# Autodesk Inventor assembly: one side of drive
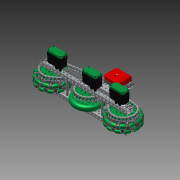
[picture p0: Inventor's stored thumbnail of the model, 180x180]
Saved by Autodesk Inventor 2014 SP1 (Build 180222100, 222)
## iProperties
Created: 2014-03-07
Part Number: one side of drive
Document SubType Name: Assembly
Designer: Ryan
Author: Ryan
## Documents named in this file (25)
- C:\Users\Ryan\Desktop\sw\toss up 5th A bot\drive\one side of drive.iam
- C:\Users\Ryan\Desktop\sw\lib\Aperture VEX CAD Library\Metal\C Channel\2 x 25.ipt
- C:\Users\Ryan\Desktop\sw\lib\Aperture VEX CAD Library\Bearing Blocks\Bearing Block with screws.iam
- C:\Users\Ryan\Desktop\sw\toss up 5th A bot\drive\wheel assembly.iam
- C:\Users\Ryan\Desktop\sw\toss up 5th A bot\drive\varsity wheel with sprocket.iam
- C:\Users\Ryan\Desktop\sw\lib\Aperture VEX CAD Library\Standoffs\BEAM-2000.ipt
- C:\Users\Ryan\Desktop\sw\lib\Aperture VEX CAD Library\Metal\C Channel\5 x 5.ipt
- C:\Users\Ryan\Desktop\sw\lib\Super Sonic Sparks VEX CAD Library\Motors & Sensors\Optical Shaft (Quadrature) Encoder.iam
- C:\Users\Ryan\Desktop\sw\lib\Aperture VEX CAD Library\Spacers\SPACER-0500-0125.ipt
- C:\Users\Ryan\Desktop\sw\lib\Aperture VEX CAD Library\Hardware\8-32\8-32_.375.ipt
- C:\Users\Ryan\Desktop\sw\lib\Aperture VEX CAD Library\Hardware\8-32\8-32 nylock.ipt
- C:\Users\Ryan\Desktop\sw\lib\Aperture VEX CAD Library\Hardware\8-32\8-32_1.500.ipt
- C:\Users\Ryan\Desktop\sw\lib\Aperture VEX CAD Library\Spacers\SPACER-0500-0500.ipt
- C:\Users\Ryan\Desktop\sw\lib\Aperture VEX CAD Library\Spacers\SPACER-0500-0375.ipt
- C:\Users\Ryan\Desktop\sw\lib\Aperture VEX CAD Library\Sprockets\green\High Strength 12-Tooth Sprocket.ipt
- C:\Users\Ryan\Desktop\sw\lib\Aperture VEX CAD Library\Bearing Blocks\Bearing Block.ipt
- C:\Users\Ryan\Desktop\sw\lib\Aperture VEX CAD Library\Hardware\8-32\8-32_.500.ipt
- C:\Users\Ryan\Desktop\sw\lib\Aperture VEX CAD Library\Hardware\Shaft Collar.ipt
- C:\Users\Ryan\Desktop\sw\lib\Aperture VEX CAD Library\Bearing Blocks\Pillow Block.ipt
- C:\Users\Ryan\Desktop\sw\lib\Aperture VEX CAD Library\Spacers\thin\SPACER-0320-0125.ipt
- C:\Users\Ryan\Desktop\sw\lib\Super Sonic Sparks VEX CAD Library\Motors & Sensors\2-Wire Motor 393-Without Wire.iam
- C:\Users\Ryan\Desktop\sw\lib\Aperture VEX CAD Library\Hardware\6-32\6-32_.250.ipt
- C:\Users\Ryan\Desktop\sw\lib\Aperture VEX CAD Library\Shaft\3.7 in shaft.ipt
- C:\Users\Ryan\Desktop\sw\lib\Aperture VEX CAD Library\Sprockets\HS Sprockets\High strength Chain Link.ipt
- C:\Users\Ryan\Desktop\sw\toss up 5th A bot\drive\one side of drive\Design Accelerator\V-Belt transmission1.iam
## Components (178 placed, 24 different names)
1. 2 x 25:1 — Mate:1, Mate:2, Mate:3, Mate:4, Mate:11, Mate:12, Mate:13, Mate:14, Mate:15, Mate:16, Flush:1, Flush:2, Mate:104, Angle:1, Mate:105, Mate:118, Mate:120, Mate:124, Mate:125
2. wheel assembly:1 [sub-assembly] — Mate:5, Mate:20, Mate:92
3. wheel assembly:2 [sub-assembly] — Mate:7, Mate:18, Mate:78
4. varsity wheel with sprocket:1 [sub-assembly] — Mate:10, Mate:19, Flush:4
5. BEAM-2000:1 — Mate:11, Mate:12, Mate:13, Mate:115, Mate:117
6. BEAM-2000:2 — Mate:14, Mate:15, Mate:16, Mate:17, Mate:119, Mate:121
7. 2 x 25:2 — Mate:17, Flush:1, Flush:2, Flush:3, Mate:77, Mate:79, Mate:80, Mate:84, Mate:86, Mate:88, Mate:89, Mate:90, Mate:91, Mate:93, Mate:95, Mate:97, Mate:101, Mate:102, Flush:5, Mate:106, Mate:107, Mate:108, Mate:109, Mate:110, Mate:111, Mate:113, Mate:116, Mate:122, Mate:127, Mate:128, Mate:129, Mate:133
8. 5 x 5:1 — Flush:3, Mate:22, Mate:23, Mate:24, Mate:26, Mate:27, Mate:31, Mate:34, Mate:36, Mate:41, Mate:45, Mate:47, Mate:49, Mate:102, Flush:5, Angle:2
9. Optical Shaft (Quadrature) Encoder:1 [sub-assembly] — Mate:22, Mate:23, Mate:24, Mate:25, Mate:33, Mate:44, Mate:46, Mate:136, Flush:7, Mate:137
10. 8-32_1.500:1 — Mate:34, Mate:36, Mate:42, Mate:43
11. SPACER-0500-0500:1 — Mate:37, Mate:38, Mate:39, Mate:43
12. SPACER-0500-0500:2 — Mate:37, Mate:38, Mate:40
13. SPACER-0500-0375:1 — Mate:39, Mate:40, Mate:41, Mate:42
14. High Strength 12-Tooth Sprocket:1 — Mate:44, Flush:4, Mate:52, Mate:53, Mate:139
15. Bearing Block:1 — Mate:45, Mate:46, Mate:47, Mate:48, Mate:50, Mate:75
16. Shaft Collar:1 — Mate:52, Mate:53, Mate:54, Mate:55
17. SPACER-0500-0500:3 — Mate:54, Mate:55, Mate:56, Mate:57, Mate:76
18. SPACER-0500-0500:4 — Mate:56, Mate:57, Mate:58, Mate:61, Mate:62
19. Pillow Block:1 — Mate:58, Mate:70, Mate:71, Mate:72, Mate:103, Angle:1, Mate:105
20. SPACER-0320-0125:1 — Mate:61, Mate:62, Mate:63, Mate:64
21. SPACER-0320-0125:2 — Mate:63, Mate:64
22. SPACER-0500-0375:2 — Mate:75, Mate:76
23. 2-Wire Motor 393-Without Wire:1 [sub-assembly] — Mate:84, Mate:85, Mate:86, Mate:87
24. Bearing Block:2 — Mate:77, Mate:78, Mate:79, Mate:81, Mate:83, Mate:85
25. 8-32_.375:6 — Mate:106, Mate:107, Mate:108, Mate:114
26. 8-32_.375:7 — Mate:109, Mate:110, Mate:111, Mate:112
27. 8-32 nylock:16 — Mate:112, Mate:113, Flush:6
28. 8-32 nylock:17 — Mate:114, Flush:6
29. 8-32_.375:8 — Mate:115, Mate:116
30. 8-32_.375:9 — Mate:117, Mate:118
31. 8-32_.375:10 — Mate:119, Mate:120
32. 8-32_.375:11 — Mate:121, Mate:122
33. 3.7 in shaft:1 — Mate:136, Flush:7, Mate:137
34. V-Belt transmission:1 [sub-assembly]
35. Bearing Block with screws:1 [sub-assembly] — Mate:1, Mate:2, Mate:3, Mate:4, Mate:5, Mate:20, Mate:123, Mate:126
36. 8-32 nylock:19 — Mate:125, Mate:126
37. 8-32 nylock:18 — Mate:123, Mate:124
38. Bearing Block with screws:2 [sub-assembly] — Mate:10, Mate:19
39. 8-32 nylock:20
40. 8-32 nylock:22
41. Bearing Block with screws:3 [sub-assembly] — Mate:7, Mate:18
42. 8-32 nylock:21
43. 8-32 nylock:23
44. SPACER-0500-0125:1 — Mate:25, Mate:26, Mate:27, Mate:30, Mate:32
45. 8-32_.375:2 — Mate:30, Mate:31
46. 8-32 nylock:1 — Mate:32, Mate:33
47. SPACER-0500-0125:2
48. 8-32_.375:3
49. 8-32 nylock:2
50. 8-32_.500:1 — Mate:48, Mate:49, Mate:51
51. 8-32 nylock:3 — Mate:50, Mate:51
52. 8-32_.500:2
53. 8-32 nylock:4
54. 8-32_.500:3 — Mate:80, Mate:81, Mate:82
55. 8-32 nylock:7 — Mate:82, Mate:83
56. 6-32_.250:1 — Mate:87, Mate:88
57. 8-32_.500:4
58. 8-32 nylock:8
59. 6-32_.250:2
60. 8-32_.375:4 — Mate:71, Mate:72
61. SPACER-0500-0500:6 — Mate:65, Mate:66, Mate:103
62. SPACER-0500-0500:7 — Mate:65, Mate:66, Mate:67, Mate:68, Mate:70
63. SPACER-0500-0500:5 — Mate:67, Mate:68, Mate:74
64. 8-32 nylock:5 — Mate:74, Mate:104
65. 8-32_.375:5
66. SPACER-0500-0500:8
67. SPACER-0500-0500:9
68. SPACER-0500-0500:10
69. 8-32 nylock:13
70. 2-Wire Motor 393-Without Wire:3 [sub-assembly] — Mate:93, Mate:94, Mate:95, Mate:100
71. Bearing Block:4 — Mate:89, Mate:90, Mate:91, Mate:92, Mate:94, Mate:96, Mate:98
72. 2-Wire Motor 393-Without Wire:4 [sub-assembly]
73. Bearing Block:5
74. 8-32_.375:12 — Mate:127, Mate:128, Mate:129
75. 8-32_.375:13 — Mate:134, Mate:135
76. SPACER-0500-0375:4 — Mate:134, Mate:135
77. SPACER-0500-0375:3 — Mate:133
78. 8-32_.375:14
79. 8-32_.375:15
80. SPACER-0500-0375:5
81. SPACER-0500-0375:6
82. High strength Chain Link:1 — Mate:139, Angle:2
83. High strength Chain Link:2
84. High strength Chain Link:3
85. High strength Chain Link:4
86. High strength Chain Link:5
87. High strength Chain Link:6
88. High strength Chain Link:7
89. High strength Chain Link:8
90. High strength Chain Link:9
91. High strength Chain Link:10
92. High strength Chain Link:11
93. High strength Chain Link:12
94. High strength Chain Link:13
95. High strength Chain Link:14
96. High strength Chain Link:15
97. High strength Chain Link:16
98. High strength Chain Link:17
99. High strength Chain Link:18
100. High strength Chain Link:19
101. High strength Chain Link:20
102. High strength Chain Link:21
103. High strength Chain Link:22
104. High strength Chain Link:23
105. High strength Chain Link:24
106. High strength Chain Link:25
107. High strength Chain Link:26
108. High strength Chain Link:27
109. High strength Chain Link:28
110. High strength Chain Link:29
111. High strength Chain Link:30
112. High strength Chain Link:31
113. High strength Chain Link:32
114. High strength Chain Link:33
115. High strength Chain Link:34
116. High strength Chain Link:35
117. High strength Chain Link:36
118. High strength Chain Link:37
119. High strength Chain Link:38
120. High strength Chain Link:39
121. High strength Chain Link:40
122. High strength Chain Link:41
123. High strength Chain Link:42
124. High strength Chain Link:43
125. High strength Chain Link:44
126. High strength Chain Link:45
127. High strength Chain Link:46
128. High strength Chain Link:47
129. High strength Chain Link:48
130. High strength Chain Link:49
131. High strength Chain Link:50
132. High strength Chain Link:51
133. High strength Chain Link:52
134. High strength Chain Link:53
135. High strength Chain Link:54
136. High strength Chain Link:55
137. High strength Chain Link:56
138. High strength Chain Link:57
139. High strength Chain Link:58
140. High strength Chain Link:59
141. High strength Chain Link:60
142. High strength Chain Link:61
143. High strength Chain Link:62
144. High strength Chain Link:63
145. High strength Chain Link:64
146. High strength Chain Link:65
147. High strength Chain Link:66
148. High strength Chain Link:67
149. High strength Chain Link:68
150. High strength Chain Link:69
151. High strength Chain Link:70
152. High strength Chain Link:71
153. High strength Chain Link:72
154. High strength Chain Link:73
155. High strength Chain Link:74
156. High strength Chain Link:75
157. High strength Chain Link:76
158. High strength Chain Link:77
159. High strength Chain Link:78
160. High strength Chain Link:79
161. High strength Chain Link:80
162. High strength Chain Link:81
163. High strength Chain Link:82
164. High strength Chain Link:83
165. High strength Chain Link:84
166. High strength Chain Link:85
167. 6-32_.250:5 — Mate:100, Mate:101
168. 8-32 nylock:11 — Mate:98, Mate:99
169. 8-32_.500:7 — Mate:96, Mate:97, Mate:99
170. 6-32_.250:6
171. 8-32 nylock:12
172. 8-32_.500:8
173. 6-32_.250:7
174. 8-32 nylock:14
175. 8-32_.500:9
176. 6-32_.250:8
177. 8-32 nylock:15
178. 8-32_.500:10
## Component patterns: (3 elements, first: Bearing Block with screws:1 + 8-32 nylock:19 + 8-32 nylock:18), (2 elements, first: SPACER-0500-0125:1 + 8-32_.375:2 + 8-32 nylock:1), (2 elements, first: 8-32_.500:1 + 8-32 nylock:3), (2 elements, first: 8-32_.500:3 + 8-32 nylock:7 + 6-32_.250:1), (2 elements, first: 8-32_.375:4 + SPACER-0500-0500:6 + SPACER-0500-0500:7 + SPACER-0500-0500:5 + 8-32 nylock:5), (2 elements, first: 2-Wire Motor 393-Without Wire:3 + Bearing Block:4), (2 elements, first: 8-32_.375:12 + 8-32_.375:13 + SPACER-0500-0375:4 + SPACER-0500-0375:3), (85 elements, first: High strength Chain Link:1), (2 elements, first: 6-32_.250:5 + 8-32 nylock:11 + 8-32_.500:7), Component Pattern 7:2 (2 elements)
## Relationships (136: Mate 127, Flush 7, Angle 2)
- Mate:1: 2 x 25:1 ↔ Bearing Block with screws:1
- Mate:2 (2.3114 mm): 2 x 25:1 ↔ Bearing Block with screws:1
- Mate:3 (2.3114 mm): 2 x 25:1 ↔ Bearing Block with screws:1
- Mate:4 (2.3114 mm): 2 x 25:1 ↔ Bearing Block with screws:1
- Mate:5: wheel assembly:1 ↔ Bearing Block with screws:1
- Mate:7: wheel assembly:2 ↔ Bearing Block with screws:3
- Mate:10: varsity wheel with sprocket:1 ↔ Bearing Block with screws:2
- Mate:11: 2 x 25:1 ↔ BEAM-2000:1
- Mate:12 (2.3114 mm): 2 x 25:1 ↔ BEAM-2000:1
- Mate:13 (2.3114 mm): 2 x 25:1 ↔ BEAM-2000:1
- Mate:14: 2 x 25:1 ↔ BEAM-2000:2
- Mate:15 (2.3114 mm): 2 x 25:1 ↔ BEAM-2000:2
- Mate:16 (2.3114 mm): 2 x 25:1 ↔ BEAM-2000:2
- Mate:17: BEAM-2000:2 ↔ 2 x 25:2
- Flush:1: 2 x 25:1 ↔ 2 x 25:2
- Mate:18: wheel assembly:2 ↔ Bearing Block with screws:3
- Mate:19: varsity wheel with sprocket:1 ↔ Bearing Block with screws:2
- Mate:20: wheel assembly:1 ↔ Bearing Block with screws:1
- Flush:2: 2 x 25:1 ↔ 2 x 25:2
- Flush:3: 2 x 25:2 ↔ 5 x 5:1
- Mate:22 (2.3114 mm): 5 x 5:1 ↔ Optical Shaft (Quadrature) Encoder:1
- Mate:23 (3.175 mm): 5 x 5:1 ↔ Optical Shaft (Quadrature) Encoder:1
- Mate:24 (-10.3886 mm): 5 x 5:1 ↔ Optical Shaft (Quadrature) Encoder:1
- Mate:25: Optical Shaft (Quadrature) Encoder:1 ↔ SPACER-0500-0125:1
- Mate:26 (2.3114 mm): 5 x 5:1 ↔ SPACER-0500-0125:1
- Mate:27 (2.3114 mm): 5 x 5:1 ↔ SPACER-0500-0125:1
- Mate:30: SPACER-0500-0125:1 ↔ 8-32_.375:2
- Mate:31: 5 x 5:1 ↔ 8-32_.375:2
- Mate:32: SPACER-0500-0125:1 ↔ 8-32 nylock:1
- Mate:33: Optical Shaft (Quadrature) Encoder:1 ↔ 8-32 nylock:1
- Mate:34 (2.3114 mm): 5 x 5:1 ↔ 8-32_1.500:1
- Mate:36 (2.3114 mm): 5 x 5:1 ↔ 8-32_1.500:1
- Mate:37: SPACER-0500-0500:1 ↔ SPACER-0500-0500:2
- Mate:38: SPACER-0500-0500:1 ↔ SPACER-0500-0500:2
- Mate:39: SPACER-0500-0500:1 ↔ SPACER-0500-0375:1
- Mate:40: SPACER-0500-0500:2 ↔ SPACER-0500-0375:1
- Mate:41: 5 x 5:1 ↔ SPACER-0500-0375:1
- Mate:42: 8-32_1.500:1 ↔ SPACER-0500-0375:1
- Mate:43: 8-32_1.500:1 ↔ SPACER-0500-0500:1
- Mate:44: Optical Shaft (Quadrature) Encoder:1 ↔ High Strength 12-Tooth Sprocket:1
- Mate:45: 5 x 5:1 ↔ Bearing Block:1
- Mate:46: Optical Shaft (Quadrature) Encoder:1 ↔ Bearing Block:1
- Mate:47 (2.3114 mm): 5 x 5:1 ↔ Bearing Block:1
- Mate:48: Bearing Block:1 ↔ 8-32_.500:1
- Mate:49: 5 x 5:1 ↔ 8-32_.500:1
- Mate:50: Bearing Block:1 ↔ 8-32 nylock:3
- Mate:51: 8-32_.500:1 ↔ 8-32 nylock:3
- Flush:4: varsity wheel with sprocket:1 ↔ High Strength 12-Tooth Sprocket:1
- Mate:52: High Strength 12-Tooth Sprocket:1 ↔ Shaft Collar:1
- Mate:53: High Strength 12-Tooth Sprocket:1 ↔ Shaft Collar:1
- Mate:54: Shaft Collar:1 ↔ SPACER-0500-0500:3
- Mate:55: Shaft Collar:1 ↔ SPACER-0500-0500:3
- Mate:56: SPACER-0500-0500:3 ↔ SPACER-0500-0500:4
- Mate:57: SPACER-0500-0500:3 ↔ SPACER-0500-0500:4
- Mate:58: SPACER-0500-0500:4 ↔ Pillow Block:1
- Mate:61: SPACER-0500-0500:4 ↔ SPACER-0320-0125:1
- Mate:62: SPACER-0500-0500:4 ↔ SPACER-0320-0125:1
- Mate:63: SPACER-0320-0125:1 ↔ SPACER-0320-0125:2
- Mate:64: SPACER-0320-0125:1 ↔ SPACER-0320-0125:2
- Mate:65: SPACER-0500-0500:6 ↔ SPACER-0500-0500:7
- Mate:66: SPACER-0500-0500:6 ↔ SPACER-0500-0500:7
- Mate:67: SPACER-0500-0500:7 ↔ SPACER-0500-0500:5
- Mate:68: SPACER-0500-0500:7 ↔ SPACER-0500-0500:5
- Mate:70: Pillow Block:1 ↔ SPACER-0500-0500:7
- Mate:71: Pillow Block:1 ↔ 8-32_.375:4
- Mate:72: Pillow Block:1 ↔ 8-32_.375:4
- Mate:74: SPACER-0500-0500:5 ↔ 8-32 nylock:5
- Mate:75: Bearing Block:1 ↔ SPACER-0500-0375:2
- Mate:76: SPACER-0500-0500:3 ↔ SPACER-0500-0375:2
- Mate:77: 2 x 25:2 ↔ Bearing Block:2
- Mate:78: wheel assembly:2 ↔ Bearing Block:2
- Mate:79 (2.3114 mm): 2 x 25:2 ↔ Bearing Block:2
- Mate:80: 2 x 25:2 ↔ 8-32_.500:3
- Mate:81: Bearing Block:2 ↔ 8-32_.500:3
- Mate:82: 8-32_.500:3 ↔ 8-32 nylock:7
- Mate:83: Bearing Block:2 ↔ 8-32 nylock:7
- Mate:84: 2 x 25:2 ↔ 2-Wire Motor 393-Without Wire:1
- Mate:85: 2-Wire Motor 393-Without Wire:1 ↔ Bearing Block:2
- Mate:86 (2.3114 mm): 2 x 25:2 ↔ 2-Wire Motor 393-Without Wire:1
- Mate:87: 2-Wire Motor 393-Without Wire:1 ↔ 6-32_.250:1
- Mate:88: 2 x 25:2 ↔ 6-32_.250:1
- Mate:89: 2 x 25:2 ↔ Bearing Block:4
- Mate:90 (2.3114 mm): 2 x 25:2 ↔ Bearing Block:4
- Mate:91 (2.3114 mm): 2 x 25:2 ↔ Bearing Block:4
- Mate:92: wheel assembly:1 ↔ Bearing Block:4
- Mate:93: 2 x 25:2 ↔ 2-Wire Motor 393-Without Wire:3
- Mate:94: 2-Wire Motor 393-Without Wire:3 ↔ Bearing Block:4
- Mate:95 (2.3114 mm): 2 x 25:2 ↔ 2-Wire Motor 393-Without Wire:3
- Mate:96: Bearing Block:4 ↔ 8-32_.500:7
- Mate:97: 2 x 25:2 ↔ 8-32_.500:7
- Mate:98: Bearing Block:4 ↔ 8-32 nylock:11
- Mate:99: 8-32 nylock:11 ↔ 8-32_.500:7
- Mate:100: 2-Wire Motor 393-Without Wire:3 ↔ 6-32_.250:5
- Mate:101: 2 x 25:2 ↔ 6-32_.250:5
- Mate:102: 2 x 25:2 ↔ 5 x 5:1
- Mate:103: Pillow Block:1 ↔ SPACER-0500-0500:6
- Mate:104: 2 x 25:1 ↔ 8-32 nylock:5
- Angle:1 (180 deg): 2 x 25:1 ↔ Pillow Block:1
- Mate:105 (2.3114 mm): 2 x 25:1 ↔ Pillow Block:1
- Flush:5: 2 x 25:2 ↔ 5 x 5:1
- Mate:106: 2 x 25:2 ↔ 8-32_.375:6
- Mate:107 (2.3114 mm): 2 x 25:2 ↔ 8-32_.375:6
- Mate:108 (2.3114 mm): 2 x 25:2 ↔ 8-32_.375:6
- Mate:109 (2.3114 mm): 2 x 25:2 ↔ 8-32_.375:7
- Mate:110 (2.3114 mm): 2 x 25:2 ↔ 8-32_.375:7
- Mate:111: 2 x 25:2 ↔ 8-32_.375:7
- Mate:112: 8-32_.375:7 ↔ 8-32 nylock:16
- Mate:113 (2.3368 mm): 2 x 25:2 ↔ 8-32 nylock:16
- Mate:114: 8-32_.375:6 ↔ 8-32 nylock:17
- Flush:6: 8-32 nylock:16 ↔ 8-32 nylock:17
- Mate:115: BEAM-2000:1 ↔ 8-32_.375:8
- Mate:116: 2 x 25:2 ↔ 8-32_.375:8
- Mate:117: BEAM-2000:1 ↔ 8-32_.375:9
- Mate:118: 2 x 25:1 ↔ 8-32_.375:9
- Mate:119: BEAM-2000:2 ↔ 8-32_.375:10
- Mate:120: 2 x 25:1 ↔ 8-32_.375:10
- Mate:121: BEAM-2000:2 ↔ 8-32_.375:11
- Mate:122: 2 x 25:2 ↔ 8-32_.375:11
- Mate:123: Bearing Block with screws:1 ↔ 8-32 nylock:18
- Mate:124: 2 x 25:1 ↔ 8-32 nylock:18
- Mate:125: 2 x 25:1 ↔ 8-32 nylock:19
- Mate:126: Bearing Block with screws:1 ↔ 8-32 nylock:19
- Mate:127 (2.3114 mm): 2 x 25:2 ↔ 8-32_.375:12
- Mate:128 (2.3114 mm): 2 x 25:2 ↔ 8-32_.375:12
- Mate:129: 2 x 25:2 ↔ 8-32_.375:12
- [Mate]: SPACER-0500-0375:4 ↔ SPACER-0500-0375:3
- [Mate]: SPACER-0500-0375:4 ↔ SPACER-0500-0375:3
- [Mate]: 8-32_.375:12 ↔ SPACER-0500-0375:4
- Mate:133: 2 x 25:2 ↔ SPACER-0500-0375:3
- Mate:134: 8-32_.375:13 ↔ SPACER-0500-0375:4
- Mate:135: 8-32_.375:13 ↔ SPACER-0500-0375:4
- Mate:136: Optical Shaft (Quadrature) Encoder:1 ↔ 3.7 in shaft:1
- Flush:7: Optical Shaft (Quadrature) Encoder:1 ↔ 3.7 in shaft:1
- Mate:137: Optical Shaft (Quadrature) Encoder:1 ↔ 3.7 in shaft:1
- Mate:139: High Strength 12-Tooth Sprocket:1 ↔ High strength Chain Link:1
- Angle:2 (133 deg): 5 x 5:1 ↔ High strength Chain Link:1
## Named parameters: q = 2.3114 mm, d177_d18 = 0 mm
